# Autodesk Inventor assembly: Ensamblaje proyecto
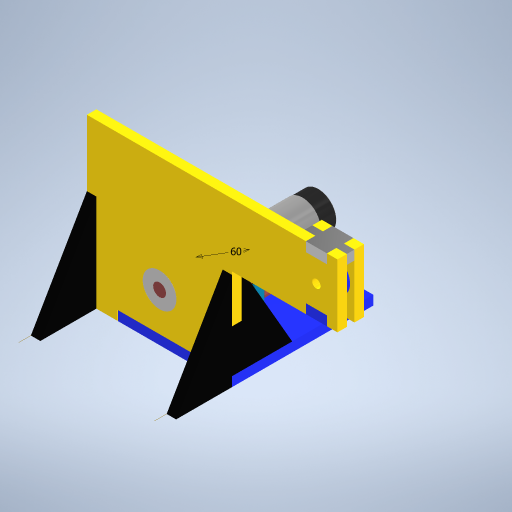
[picture p0: Inventor's stored thumbnail of the model, 512x512]
Saved by Autodesk Inventor 2024 (Build 280153000, 153)
## iProperties
Created: 2024-05-28
Part Number: Ensamblaje proyecto
Document SubType Name: Assembly
Designer: Elena Portas
Author: Elena Portas
## Documents named in this file (14)
- C:\Ricardo\ROBOTICA\ProyectoFinal\CAD\Ensamblaje proyecto.iam
- C:\Ricardo\ROBOTICA\ProyectoFinal\CAD\Balero.ipt
- C:\Ricardo\ROBOTICA\ProyectoFinal\CAD\Polea.ipt
- C:\Ricardo\ROBOTICA\ProyectoFinal\CAD\SoporteMotor.ipt
- C:\Ricardo\ROBOTICA\ProyectoFinal\CAD\Soporte pared.ipt
- C:\Ricardo\ROBOTICA\ProyectoFinal\CAD\SoporteSoporte.ipt
- C:\Ricardo\ROBOTICA\ProyectoFinal\CAD\Base.ipt
- C:\Ricardo\ROBOTICA\ProyectoFinal\CAD\SoporteCarrete.ipt
- C:\Ricardo\ROBOTICA\ProyectoFinal\CAD\Polulu v16.ipt
- C:\Ricardo\ROBOTICA\ProyectoFinal\CAD\CarreteAspas ensanchadas.ipt
- C:\Ricardo\ROBOTICA\ProyectoFinal\CAD\Balero6201.ipt
- C:\Ricardo\ROBOTICA\ProyectoFinal\CAD\SoporteBaleroSuperior.ipt
- C:\Ricardo\ROBOTICA\ProyectoFinal\CAD\SoportePoleaFrontal.ipt
- C:\Ricardo\ROBOTICA\ProyectoFinal\CAD\SoportePoleaInferior.ipt
## Components (15 placed, 13 different names)
1. Balero608:1 — Nivelación:3, De rotación:2, Coincidencia:23, Cilíndrica:6
2. Polea:1 — Nivelación:3, De rotación:2
3. SoporteMotor:1 — Coincidencia:21, Cilíndrica:5, Coincidencia:22
4. Soporte pared:1 — Coincidencia:1, Coincidencia:2, Coincidencia:3, Coincidencia:4, Coincidencia:5, Coincidencia:6, Nivelación:1, Nivelación:2, Coincidencia:7, Nivelación:6, Cilíndrica:3, Coincidencia:23, Cilíndrica:6, Coincidencia:25, Coincidencia:26, Nivelación:9
5. SoporteSoporte:1 — Coincidencia:4, Coincidencia:5, Coincidencia:6
6. SoporteSoporte:2 — Coincidencia:1, Coincidencia:2, Coincidencia:3
7. Base:1 — Nivelación:1, Nivelación:2, Coincidencia:7, Nivelación:5, Coincidencia:14, Coincidencia:15, Coincidencia:22
8. SoporteCarrete:2 — Nivelación:5, Coincidencia:14, Coincidencia:15
9. Polulu v16:1 — Cilíndrica:4, Coincidencia:18, Coincidencia:19, Coincidencia:21, Cilíndrica:5
10. CarreteAspas ensanchadas:1 — Coincidencia:16, Cilíndrica:1, Coincidencia:17, Cilíndrica:2, Cilíndrica:4, Coincidencia:18, Coincidencia:19
11. Balero6201:1 — Coincidencia:16, Cilíndrica:1, Nivelación:6, Cilíndrica:3
12. Balero6201:2 — Coincidencia:17, Cilíndrica:2
13. SoportePoleaSuperior:1 — Nivelación:8, Coincidencia:25, Coincidencia:26, Nivelación:9, Coincidencia:27, Coincidencia:28
14. SoportePoleaFrontal:1 — Nivelación:8, Coincidencia:27, Coincidencia:28, Coincidencia:29, Nivelación:31, Coincidencia:30
15. SoportePoleaInferior:1 — Coincidencia:29, Nivelación:31, Coincidencia:30
## Relationships (37: Mate 22, Flush 8, CylindricalJoint 6, RevoluteJoint 1)
- Coincidencia:1 [Mate]: Soporte pared:1 ↔ SoporteSoporte:2
- Coincidencia:2 [Mate]: Soporte pared:1 ↔ SoporteSoporte:2
- Coincidencia:3 [Mate]: Soporte pared:1 ↔ SoporteSoporte:2
- Coincidencia:4 [Mate]: Soporte pared:1 ↔ SoporteSoporte:1
- Coincidencia:5 [Mate]: Soporte pared:1 ↔ SoporteSoporte:1
- Coincidencia:6 [Mate]: Soporte pared:1 ↔ SoporteSoporte:1
- Nivelación:1 [Flush]: Soporte pared:1 ↔ Base:1
- Nivelación:2 [Flush]: Soporte pared:1 ↔ Base:1
- Coincidencia:7 [Mate]: Soporte pared:1 ↔ Base:1
- Nivelación:3 [Flush]: Balero608:1 ↔ Polea:1
- De rotación:2 [RevoluteJoint]: Balero608:1 ↔ Polea:1
- Nivelación:5 [Flush]: Base:1 ↔ SoporteCarrete:2
- Coincidencia:14 [Mate]: Base:1 ↔ SoporteCarrete:2
- Coincidencia:15 [Mate]: Base:1 ↔ SoporteCarrete:2
- Coincidencia:16 [Mate]: CarreteAspas ensanchadas:1 ↔ Balero6201:1
- Cilíndrica:1 [CylindricalJoint]: CarreteAspas ensanchadas:1 ↔ Balero6201:1
- Coincidencia:17 [Mate]: CarreteAspas ensanchadas:1 ↔ Balero6201:2
- Cilíndrica:2 [CylindricalJoint]: CarreteAspas ensanchadas:1 ↔ Balero6201:2
- Nivelación:6 [Flush]: Soporte pared:1 ↔ Balero6201:1
- Cilíndrica:3 [CylindricalJoint]: Soporte pared:1 ↔ Balero6201:1
- Cilíndrica:4 [CylindricalJoint]: Polulu v16:1 ↔ CarreteAspas ensanchadas:1
- Coincidencia:18 [Mate]: Polulu v16:1 ↔ CarreteAspas ensanchadas:1
- Coincidencia:19 [Mate]: Polulu v16:1 ↔ CarreteAspas ensanchadas:1
- Coincidencia:21 [Mate]: SoporteMotor:1 ↔ Polulu v16:1
- Cilíndrica:5 [CylindricalJoint]: SoporteMotor:1 ↔ Polulu v16:1
- Coincidencia:22 [Mate]: SoporteMotor:1 ↔ Base:1
- Coincidencia:23 [Mate]: Balero608:1 ↔ Soporte pared:1
- Cilíndrica:6 [CylindricalJoint]: Balero608:1 ↔ Soporte pared:1
- Nivelación:8 [Flush]: SoportePoleaSuperior:1 ↔ SoportePoleaFrontal:1
- Coincidencia:25 [Mate]: Soporte pared:1 ↔ SoportePoleaSuperior:1
- Coincidencia:26 [Mate]: Soporte pared:1 ↔ SoportePoleaSuperior:1
- Nivelación:9 [Flush]: Soporte pared:1 ↔ SoportePoleaSuperior:1
- Coincidencia:27 [Mate]: SoportePoleaSuperior:1 ↔ SoportePoleaFrontal:1
- Coincidencia:28 [Mate]: SoportePoleaSuperior:1 ↔ SoportePoleaFrontal:1
- Coincidencia:29 [Mate]: SoportePoleaFrontal:1 ↔ SoportePoleaInferior:1
- Nivelación:31 [Flush]: SoportePoleaFrontal:1 ↔ SoportePoleaInferior:1
- Coincidencia:30 [Mate]: SoportePoleaFrontal:1 ↔ SoportePoleaInferior:1
